# Autodesk Inventor assembly: ASY NVPH-500 hopper support
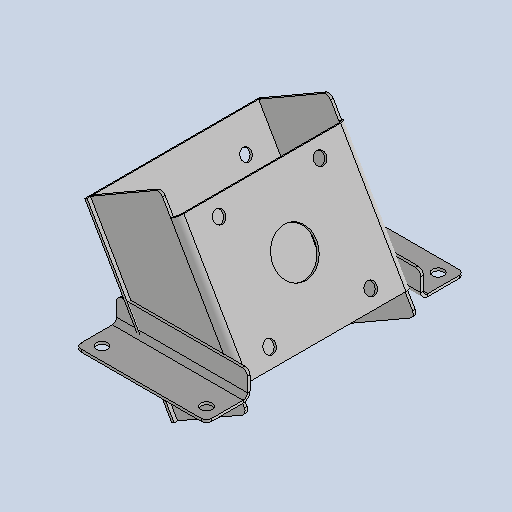
[picture p0: Inventor's stored thumbnail of the model, 512x512]
Saved by Autodesk Inventor 2025.1 (Build 291241020, 241B)
## iProperties
Created: 2025-02-25
Part Number: ASY NVPH-500 hopper support
Document SubType Name: Assembly
Designer: user
Author: user
## Documents named in this file (4)
- C:\Users\user\YandexDisk-badmisterfox\home pc\Inventor\NDM-VOS_powder_hopper\ASY NVPH-500 hopper support.iam
- C:\Users\user\YandexDisk-badmisterfox\home pc\Inventor\NDM-VOS_powder_hopper\NDM-VOS 777 sredder wall 7.ipt
- C:\Users\user\YandexDisk-badmisterfox\home pc\Inventor\NDM-VOS_powder_hopper\NDM-VOS 778 engine plate.ipt
- C:\Users\user\YandexDisk-badmisterfox\home pc\Inventor\NDM-VOS_powder_hopper\NDM-VOS 712 flange.ipt
## Components (4 placed, 3 different names)
1. NDM-VOS 112 sredder wall sub:1
2. NDM-VOS 778 engine plate:1
3. NDM-VOS 712 flange:1
4. NDM-VOS 712 flange:2
## Relationships (5: Mate 2, Flush 2, WeldJoint 1)
- [WeldJoint]: NDM-VOS 112 sredder wall sub:1 ↔ NDM-VOS 778 engine plate:1
- [Mate]: NDM-VOS 778 engine plate:1 ↔ NDM-VOS 712 flange:1
- [Mate]: NDM-VOS 778 engine plate:1 ↔ NDM-VOS 712 flange:2
- [Flush]: NDM-VOS 712 flange:1 ↔ NDM-VOS 712 flange:2
- [Flush]: NDM-VOS 712 flange:1 ↔ NDM-VOS 712 flange:2
